# Autodesk Inventor assembly: 1603A230_Hinge
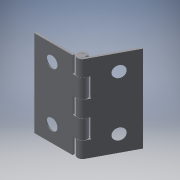
[picture p0: Inventor's stored thumbnail of the model, 180x180]
Saved by Autodesk Inventor 2019 (Build 230136000, 136)
## iProperties
Created: 2019-03-12
Part Number: 1603A230_Hinge
Document SubType Name: Assembly
Designer: User
Author: User
## Documents named in this file (4)
- C:\Robotics\CAD\COTSParts\Hinges\1603A230_Hinge.iam
- C:\Robotics\CAD\COTSParts\Hinges\1603A230_Hinge_DoorLeaf.ipt
- C:\Robotics\CAD\COTSParts\Hinges\1603A230_HingePin.ipt
- C:\Robotics\CAD\COTSParts\Hinges\1603A230_Hinge_FrameLeaf.ipt
## Components (3 placed, 3 different names)
1. 1603A230_Hinge_DoorLeaf:1 — Insert:1, Flush:1
2. 1603A230_HingePin:1 — Insert:1, Mate:1
3. 1603A230_Hinge_FrameLeaf:1 — Mate:1, Flush:1
## Relationships (3: Insert 1, Mate 1, Flush 1)
- Insert:1: 1603A230_Hinge_DoorLeaf:1 ↔ 1603A230_HingePin:1
- Mate:1: 1603A230_HingePin:1 ↔ 1603A230_Hinge_FrameLeaf:1
- Flush:1: 1603A230_Hinge_DoorLeaf:1 ↔ 1603A230_Hinge_FrameLeaf:1
